# Autodesk Inventor assembly: Assembled
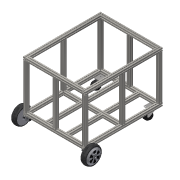
[picture p0: Inventor's stored thumbnail of the model, 180x180]
Saved by Autodesk Inventor 2019 (Build 230136000, 136)
## iProperties
Created: 2019-04-15
Part Number: Assembled
Material: 일반
Document SubType Name: Assembly
Designer: hinmo
Mass: 10081.8 g
Surface Area: 43119.5 cm^2
Volume: 3734 cm^3
Density: 2.7 g/cm^3
Author: hinmo
## Documents named in this file (7)
- C:\Users\hinmo\Documents\Inventor\Projects\2019_CapstoneDesign\Assembled.iam
- C:\Users\hinmo\Documents\Inventor\Projects\2019_CapstoneDesign\Body.iam
- C:\Users\hinmo\Documents\Inventor\Projects\2019_CapstoneDesign\SHTA16-25.iam
- C:\Users\hinmo\Documents\Inventor\Projects\2019_CapstoneDesign\SHKLMT16.iam
- C:\Users\hinmo\Documents\Inventor\Projects\2019_CapstoneDesign\Wheel_6p5in.ipt
- C:\Users\hinmo\Documents\Inventor\Projects\2019_CapstoneDesign\WJ_75.iam
- C:\Users\hinmo\Documents\Inventor\Projects\2019_CapstoneDesign\Controller.iam
## Components (10 placed, 6 different names)
1. Body:1 [sub-assembly] — 메이트:1, 메이트:2, 메이트:3, 메이트:4, 메이트:5, 메이트:6, 메이트:7, 메이트:8, 메이트:9, 메이트:13, 메이트:14, 메이트:15, 메이트:17, 메이트:18, 메이트:19, 메이트:20, 메이트:21, 메이트:22, 메이트:23, 메이트:24, 메이트:25, 메이트:26, 메이트:27
2. SHTA16-25:1 [sub-assembly] — 메이트:4, 메이트:9, 메이트:10, 각도:2, 메이트:19
3. SHTA16-25:2 [sub-assembly] — 메이트:7, 메이트:8, 메이트:11, 메이트:13, 각도:1
4. SHKLMT16:1 [sub-assembly] — 메이트:5, 메이트:16, 메이트:18
5. SHKLMT16:2 [sub-assembly] — 메이트:6, 메이트:12, 메이트:14
6. Wheel_6p5in:1 — 메이트:11, 메이트:12, 각도:1, 메이트:15
7. Wheel_6p5in:2 — 메이트:10, 메이트:16, 메이트:17, 각도:2
8. WJ_75:1 [sub-assembly] — 메이트:20, 메이트:22, 메이트:23, 메이트:24
9. WJ_75:2 [sub-assembly] — 메이트:21, 메이트:25, 메이트:26, 메이트:27, 각도:3, 접선:1
10. Controller:1 [sub-assembly]
## Relationships (31: Mate 27, Angle 3, Tangent 1)
- 메이트:1 [Mate]: Body:1
- 메이트:2 [Mate]: Body:1
- 메이트:3 [Mate]: Body:1
- 메이트:4 [Mate]: Body:1 ↔ SHTA16-25:1
- 메이트:5 [Mate]: Body:1 ↔ SHKLMT16:1
- 메이트:6 [Mate]: Body:1 ↔ SHKLMT16:2
- 메이트:7 [Mate]: Body:1 ↔ SHTA16-25:2
- 메이트:8 [Mate] (-15 mm): Body:1 ↔ SHTA16-25:2
- 메이트:9 [Mate] (-15 mm): Body:1 ↔ SHTA16-25:1
- 메이트:10 [Mate]: SHTA16-25:1 ↔ Wheel_6p5in:2
- 메이트:11 [Mate]: SHTA16-25:2 ↔ Wheel_6p5in:1
- 메이트:12 [Mate]: SHKLMT16:2 ↔ Wheel_6p5in:1
- 메이트:13 [Mate] (-15 mm): Body:1 ↔ SHTA16-25:2
- 메이트:14 [Mate] (-15 mm): Body:1 ↔ SHKLMT16:2
- 각도:1 [Angle] (0 deg): SHTA16-25:2 ↔ Wheel_6p5in:1
- 메이트:15 [Mate] (10 mm): Body:1 ↔ Wheel_6p5in:1
- 메이트:16 [Mate]: SHKLMT16:1 ↔ Wheel_6p5in:2
- 메이트:17 [Mate] (10 mm): Body:1 ↔ Wheel_6p5in:2
- 각도:2 [Angle] (0 deg): SHTA16-25:1 ↔ Wheel_6p5in:2
- 메이트:18 [Mate] (-15 mm): Body:1 ↔ SHKLMT16:1
- 메이트:19 [Mate] (-15 mm): Body:1 ↔ SHTA16-25:1
- 메이트:20 [Mate]: Body:1 ↔ WJ_75:1
- 메이트:21 [Mate]: Body:1 ↔ WJ_75:2
- 메이트:22 [Mate] (-15 mm): Body:1 ↔ WJ_75:1
- 메이트:23 [Mate] (-15 mm): Body:1 ↔ WJ_75:1
- 메이트:24 [Mate] (-15 mm): Body:1 ↔ WJ_75:1
- 메이트:25 [Mate] (-15 mm): Body:1 ↔ WJ_75:2
- 메이트:26 [Mate] (-15 mm): Body:1 ↔ WJ_75:2
- 메이트:27 [Mate] (-15 mm): Body:1 ↔ WJ_75:2
- 각도:3 [Angle] (0 deg): WJ_75:2
- 접선:1 [Tangent]: WJ_75:2
